# Autodesk Inventor assembly: Turntable-ArmConnection
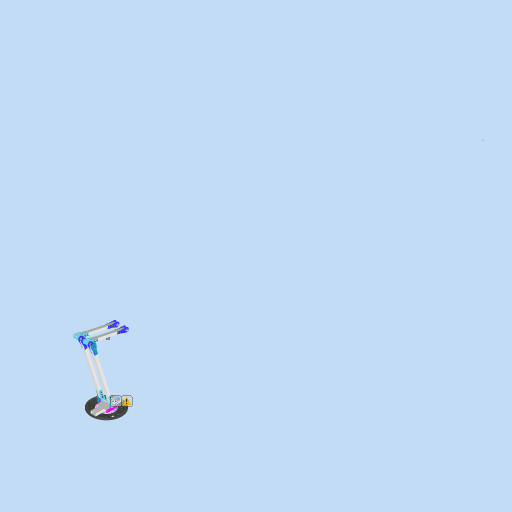
[picture p0: Inventor's stored thumbnail of the model, 512x512]
Saved by Autodesk Inventor 2024 (Build 280153000, 153)
## iProperties
Created: 2024-01-10
Part Number: Turntable-ArmConnection
Document SubType Name: Assembly
Designer: megan
Author: megan
## Documents named in this file (18)
- C:\Users\megan\OneDrive\Documents\GitHub\BehrendURCMechanical\CAD\Apparatus\Arm Base\Turntable-ArmConnection.iam
- C:\Users\megan\OneDrive\Documents\GitHub\BehrendURCMechanical\CAD\Apparatus\Arm Base\1544T3_Lubricated Turntable.ipt
- C:\Users\megan\OneDrive\Documents\GitHub\BehrendURCMechanical\CAD\Apparatus\Arm Base\2inTubeBase.ipt
- C:\Users\megan\OneDrive\Documents\GitHub\BehrendURCMechanical\CAD\Apparatus\Arm Base\1inTubeBase.ipt
- C:\Users\megan\OneDrive\Documents\GitHub\BehrendURCMechanical\CAD\Apparatus\Arm Base\ArmPlateBase.ipt
- C:\Users\megan\OneDrive\Documents\GitHub\BehrendURCMechanical\CAD\Apparatus\Arm Base\JointShaft.ipt
- C:\Users\megan\OneDrive\Documents\GitHub\BehrendURCMechanical\CAD\Chassis V3\Arm Plate2.ipt
- C:\Users\megan\OneDrive\Documents\GitHub\BehrendURCMechanical\CAD\Chassis V3\24in long 1in square tube.ipt
- C:\Users\megan\OneDrive\Documents\GitHub\BehrendURCMechanical\CAD\Chassis V3\Arm Plate3.ipt
- C:\Users\megan\OneDrive\Documents\GitHub\BehrendURCMechanical\CAD\Apparatus\Arm Base\8mmBearing.ipt
- C:\Users\megan\OneDrive\Documents\GitHub\BehrendURCMechanical\CAD\Chassis V3\Arm Plate.ipt
- C:\Users\megan\OneDrive\Documents\GitHub\BehrendURCMechanical\CAD\Chassis V3\14in long 1in square tube.ipt
- C:\Users\megan\OneDrive\Documents\GitHub\BehrendURCMechanical\CAD\Chassis V3\Bolt Nut Washer assem.iam
- C:\Users\megan\OneDrive\Documents\GitHub\BehrendURCMechanical\CAD\Apparatus\Arm Base\AP-0-02-baseAllTry2.iam
- C:\Users\megan\OneDrive\Documents\GitHub\BehrendURCMechanical\CAD\Chassis V3\90107A011_316 Stainless Steel Washer.ipt
- C:\Users\megan\OneDrive\Documents\GitHub\BehrendURCMechanical\CAD\Chassis V3\Arm Plate4.ipt
- C:\Users\megan\OneDrive\Documents\GitHub\BehrendURCMechanical\CAD\Apparatus\91290A198_Alloy Steel Socket Head Screw.ipt
- C:\Users\megan\OneDrive\Documents\GitHub\BehrendURCMechanical\CAD\Chassis V3\91831A011_18-8 Stainless Steel Nylon-Insert Locknut.ipt
## Components (75 placed, 14 different names)
1. 1544T3_Lubricated Turntable:1 — Mate:3, Mate:197, Mate:198, Mate:199, Mate:201
2. 2inTubeBase:1 — Mate:3, Mate:4, Mate:43, Mate:54, Mate:55, Mate:56, Flush:3, Flush:4, Flush:5, Mate:197, Mate:198
3. 1inTubeBase:1 — Mate:54, Mate:55, Mate:61, Mate:62, Flush:4
4. 1inTubeBase:2 — Mate:4, Mate:56, Flush:3, Mate:57, Mate:58, Mate:59, Mate:60
5. ArmPlateBase:2 — Mate:61, Mate:62, Flush:5, Mate:66
6. JointShaft:1 — Mate:22, Mate:33, Mate:36, Mate:37, Mate:63, Mate:83, Mate:84
7. arm plate:1 — Mate:22, Mate:34, Mate:73, Mate:74, Mate:142, Mate:143, Mate:150, Mate:151, Mate:152, Mate:153
8. ArmPlateBase:1 — Mate:57, Mate:58, Mate:59, Mate:60, Mate:63, Mate:65
9. 24in long 1in square tube:1 — Mate:44, Mate:45, Mate:46, Flush:2, Mate:67, Mate:68, Mate:69, Mate:70, Mate:71, Mate:72, Mate:86, Mate:200
10. 24in long 1in square tube:2 — Flush:2, Mate:49, Mate:50, Mate:51, Mate:73, Mate:74, Mate:85, Mate:204, Mate:207
11. arm plate:2 — Mate:33, Mate:34, Mate:43, Mate:44, Mate:45, Mate:46, Mate:144, Mate:145, Mate:146, Mate:147, Mate:148, Mate:149
12. 8mmBearing:1 — Mate:36, Mate:66
13. 8mmBearing:2 — Mate:37, Mate:65
14. arm plate:3 — Mate:80, Mate:81, Mate:204, Mate:207, Mate:236, Mate:237
15. arm plate:4 — Mate:49, Mate:50, Mate:51, Mate:213, Mate:262, Mate:264, Mate:266
16. arm plate:5 — Mate:67, Mate:68, Mate:69, Mate:77, Mate:78, Mate:154, Mate:155, Mate:156, Mate:157, Mate:158, Mate:168, Mate:169
17. arm plate:6 — Mate:70, Mate:71, Mate:72, Mate:79, Mate:82, Mate:161
18. 8mmBearing:4 — Mate:77, Mate:78, Mate:87
19. 8mmBearing:5 — Mate:79, Mate:82
20. 8mmBearing:6 — Mate:80, Mate:81, Mate:203, Mate:235
21. arm plate:7 — Mate:84, Mate:86
22. arm plate:8 — Mate:83, Mate:85
23. JointShaft:2 — Mate:87, Mate:93, Mate:95, Mate:97, Flush:10, Mate:203, Mate:212, Mate:226
24. 14in long 1in square tube:1 — Mate:101, Flush:7, Flush:8, Mate:106, Mate:107, Mate:110, Mate:115, Mate:116, Mate:159, Mate:227, Mate:228
25. 14in long 1in square tube:2 — Flush:8, Mate:103, Mate:104, Mate:105, Mate:108, Mate:109, Mate:112, Mate:113, Flush:9, Mate:114, Mate:160
26. arm plate:10 — Mate:93, Mate:104, Mate:105, Mate:161, Mate:170, Mate:171, Mate:172, Mate:173, Mate:174, Mate:175
27. arm plate:11 — Mate:95, Mate:101, Flush:7, Mate:158, Mate:159
28. arm plate:12 — Mate:97, Mate:103, Mate:160
29. arm plate:13 — Mate:106, Mate:107, Mate:111, Mate:115, Mate:117, Mate:124, Mate:188, Mate:189, Mate:190, Mate:191, Mate:192, Mate:193
30. arm plate:14 — Mate:108, Mate:109, Mate:114, Mate:122
31. arm plate:15 — Mate:110, Mate:111, Mate:116, Mate:120
32. arm plate:16 — Mate:112, Mate:113, Flush:9, Mate:118, Mate:182, Mate:183, Mate:184, Mate:185, Mate:186, Mate:187
33. JointShaft:3 — Mate:117, Flush:10, Mate:119, Mate:121, Mate:123, Mate:125, Flush:12
34. 8mmBearing:7 — Mate:124, Mate:125
35. 8mmBearing:8 — Mate:120, Mate:121
36. 8mmBearing:9 — Mate:118, Mate:119, Flush:12
37. 8mmBearing:10 — Mate:122, Mate:123
38. Bolt Nut Washer assem:1 [sub-assembly] — Mate:142, Mate:143
39. Bolt Nut Washer assem:2 [sub-assembly] — Mate:146, Mate:147
40. Bolt Nut Washer assem:3 [sub-assembly] — Mate:144, Mate:145
41. Bolt Nut Washer assem:4 [sub-assembly] — Mate:148, Mate:149
42. Bolt Nut Washer assem:5 [sub-assembly] — Mate:150, Mate:151
43. Bolt Nut Washer assem:6 [sub-assembly] — Mate:152, Mate:153
44. Bolt Nut Washer assem:7 [sub-assembly] — Mate:154, Mate:157
45. Bolt Nut Washer assem:8 [sub-assembly] — Mate:155, Mate:156
46. Bolt Nut Washer assem:9 [sub-assembly] — Mate:232, Mate:233
47. Bolt Nut Washer assem:10 [sub-assembly] — Mate:168, Mate:169
48. Bolt Nut Washer assem:11 [sub-assembly] — Mate:174, Mate:175
49. Bolt Nut Washer assem:13 [sub-assembly] — Mate:172, Mate:173
50. Bolt Nut Washer assem:14 [sub-assembly] — Mate:170, Mate:171
51. Bolt Nut Washer assem:15 [sub-assembly] — Mate:229, Mate:230
52. Bolt Nut Washer assem:16 [sub-assembly] — Mate:231, Mate:234
53. Bolt Nut Washer assem:17 [sub-assembly] — Mate:186, Mate:187
54. Bolt Nut Washer assem:18 [sub-assembly] — Mate:190, Mate:191
55. Bolt Nut Washer assem:19 [sub-assembly] — Mate:182, Mate:183
56. Bolt Nut Washer assem:20 [sub-assembly] — Mate:188, Mate:189
57. Bolt Nut Washer assem:21 [sub-assembly] — Mate:184, Mate:185
58. Bolt Nut Washer assem:24 [sub-assembly] — Mate:192, Mate:193
59. AP-0-02-baseAllTry2:1 [sub-assembly] — Mate:199
60. 8mmBearing:11 — Mate:212, Mate:213
61. 90107A011_316 Stainless Steel Washer:1 — Mate:240
62. 90107A011_316 Stainless Steel Washer:2 — Mate:246, Mate:247, Mate:250
63. 90107A011_316 Stainless Steel Washer:3 — Mate:243, Mate:244, Mate:245, Mate:246, Mate:249
64. arm plate:18 — Mate:226, Mate:227, Mate:228, Mate:229, Mate:230, Mate:231, Mate:232, Mate:233, Mate:234
65. arm plate:19 — Mate:235, Mate:236, Mate:237, Mate:240, Mate:243, Mate:244, Mate:245, Mate:247, Mate:248, Mate:251, Mate:252, Mate:253, Mate:255, Mate:256, Mate:258, Mate:260
66. 91290A198_Alloy Steel Socket Head Screw:1 — Mate:248, Mate:249, Mate:257, Mate:263
67. 91290A198_Alloy Steel Socket Head Screw:2 — Mate:254, Mate:255, Mate:261, Mate:267
68. 91290A198_Alloy Steel Socket Head Screw:3 — Mate:250, Mate:251, Mate:259, Mate:265
69. 90107A011_316 Stainless Steel Washer:4 — Mate:252, Mate:253, Mate:254
70. 91831A011_18-8 Stainless Steel Nylon-Insert Locknut:4 — Mate:256, Mate:257
71. 91831A011_18-8 Stainless Steel Nylon-Insert Locknut:5 — Mate:262, Mate:263
72. 91831A011_18-8 Stainless Steel Nylon-Insert Locknut:6 — Mate:260, Mate:261
73. 91831A011_18-8 Stainless Steel Nylon-Insert Locknut:7 — Mate:258, Mate:259
74. 91831A011_18-8 Stainless Steel Nylon-Insert Locknut:8 — Mate:266, Mate:267
75. 91831A011_18-8 Stainless Steel Nylon-Insert Locknut:9 — Mate:264, Mate:265
## Relationships (169: Mate 160, Flush 9)
- Mate:3: 1544T3_Lubricated Turntable:1 ↔ 2inTubeBase:1
- Mate:4: 2inTubeBase:1 ↔ 1inTubeBase:2
- Mate:22: JointShaft:1 ↔ arm plate:1
- Mate:33: JointShaft:1 ↔ arm plate:2
- Mate:34 (120.65 mm): arm plate:1 ↔ arm plate:2
- Mate:36: JointShaft:1 ↔ 8mmBearing:1
- Mate:37: JointShaft:1 ↔ 8mmBearing:2
- Mate:43 (60.325 mm): 2inTubeBase:1 ↔ arm plate:2
- Mate:44: 24in long 1in square tube:1 ↔ arm plate:2
- Mate:45: 24in long 1in square tube:1 ↔ arm plate:2
- Mate:46: 24in long 1in square tube:1 ↔ arm plate:2
- Flush:2: 24in long 1in square tube:1 ↔ 24in long 1in square tube:2
- Mate:49: 24in long 1in square tube:2 ↔ arm plate:4
- Mate:50: 24in long 1in square tube:2 ↔ arm plate:4
- Mate:51: 24in long 1in square tube:2 ↔ arm plate:4
- Mate:54: 2inTubeBase:1 ↔ 1inTubeBase:1
- Mate:55: 2inTubeBase:1 ↔ 1inTubeBase:1
- Mate:56: 2inTubeBase:1 ↔ 1inTubeBase:2
- Flush:3: 2inTubeBase:1 ↔ 1inTubeBase:2
- Mate:57: 1inTubeBase:2 ↔ ArmPlateBase:1
- Mate:58: 1inTubeBase:2 ↔ ArmPlateBase:1
- Mate:59: 1inTubeBase:2 ↔ ArmPlateBase:1
- Mate:60: 1inTubeBase:2 ↔ ArmPlateBase:1
- Mate:61: 1inTubeBase:1 ↔ ArmPlateBase:2
- Mate:62: 1inTubeBase:1 ↔ ArmPlateBase:2
- Flush:4: 2inTubeBase:1 ↔ 1inTubeBase:1
- Flush:5: 2inTubeBase:1 ↔ ArmPlateBase:2
- Mate:63: JointShaft:1 ↔ ArmPlateBase:1
- Mate:65: ArmPlateBase:1 ↔ 8mmBearing:2
- Mate:66: ArmPlateBase:2 ↔ 8mmBearing:1
- Mate:67: 24in long 1in square tube:1 ↔ arm plate:5
- Mate:68: 24in long 1in square tube:1 ↔ arm plate:5
- Mate:69: 24in long 1in square tube:1 ↔ arm plate:5
- Mate:70: 24in long 1in square tube:1 ↔ arm plate:6
- Mate:71: 24in long 1in square tube:1 ↔ arm plate:6
- Mate:72: 24in long 1in square tube:1 ↔ arm plate:6
- Mate:73: arm plate:1 ↔ 24in long 1in square tube:2
- Mate:74: arm plate:1 ↔ 24in long 1in square tube:2
- Mate:77: arm plate:5 ↔ 8mmBearing:4
- Mate:78: arm plate:5 ↔ 8mmBearing:4
- Mate:79: arm plate:6 ↔ 8mmBearing:5
- Mate:80: arm plate:3 ↔ 8mmBearing:6
- Mate:81: arm plate:3 ↔ 8mmBearing:6
- Mate:82: arm plate:6 ↔ 8mmBearing:5
- Mate:83: JointShaft:1 ↔ arm plate:8
- Mate:84: JointShaft:1 ↔ arm plate:7
- Mate:85: 24in long 1in square tube:2 ↔ arm plate:8
- Mate:86: 24in long 1in square tube:1 ↔ arm plate:7
- Mate:87: 8mmBearing:4 ↔ JointShaft:2
- Mate:93: JointShaft:2 ↔ arm plate:10
- Mate:95: JointShaft:2 ↔ arm plate:11
- Mate:97: JointShaft:2 ↔ arm plate:12
- Mate:101: 14in long 1in square tube:1 ↔ arm plate:11
- Flush:7: 14in long 1in square tube:1 ↔ arm plate:11
- Flush:8: 14in long 1in square tube:1 ↔ 14in long 1in square tube:2
- Mate:103: 14in long 1in square tube:2 ↔ arm plate:12
- Mate:104: 14in long 1in square tube:2 ↔ arm plate:10
- Mate:105: 14in long 1in square tube:2 ↔ arm plate:10
- Mate:106: 14in long 1in square tube:1 ↔ arm plate:13
- Mate:107: 14in long 1in square tube:1 ↔ arm plate:13
- Mate:108: 14in long 1in square tube:2 ↔ arm plate:14
- Mate:109: 14in long 1in square tube:2 ↔ arm plate:14
- Mate:110: 14in long 1in square tube:1 ↔ arm plate:15
- Mate:111: arm plate:13 ↔ arm plate:15
- Mate:112: 14in long 1in square tube:2 ↔ arm plate:16
- Mate:113: 14in long 1in square tube:2 ↔ arm plate:16
- Flush:9 (-2 mm): 14in long 1in square tube:2 ↔ arm plate:16
- Mate:114: 14in long 1in square tube:2 ↔ arm plate:14
- Mate:115: 14in long 1in square tube:1 ↔ arm plate:13
- Mate:116: 14in long 1in square tube:1 ↔ arm plate:15
- Mate:117: arm plate:13 ↔ JointShaft:3
- Flush:10: JointShaft:2 ↔ JointShaft:3
- Mate:118: arm plate:16 ↔ 8mmBearing:9
- Mate:119: JointShaft:3 ↔ 8mmBearing:9
- Mate:120: arm plate:15 ↔ 8mmBearing:8
- Mate:121: JointShaft:3 ↔ 8mmBearing:8
- Mate:122: arm plate:14 ↔ 8mmBearing:10
- Mate:123: JointShaft:3 ↔ 8mmBearing:10
- Mate:124: arm plate:13 ↔ 8mmBearing:7
- Mate:125: JointShaft:3 ↔ 8mmBearing:7
- Mate:142: arm plate:1 ↔ Bolt Nut Washer assem:1
- Mate:143: arm plate:1 ↔ Bolt Nut Washer assem:1
- Mate:144: arm plate:2 ↔ Bolt Nut Washer assem:3
- Mate:145: arm plate:2 ↔ Bolt Nut Washer assem:3
- Mate:146: arm plate:2 ↔ Bolt Nut Washer assem:2
- Mate:147: arm plate:2 ↔ Bolt Nut Washer assem:2
- Mate:148: arm plate:2 ↔ Bolt Nut Washer assem:4
- Mate:149: arm plate:2 ↔ Bolt Nut Washer assem:4
- Mate:150: arm plate:1 ↔ Bolt Nut Washer assem:5
- Mate:151: arm plate:1 ↔ Bolt Nut Washer assem:5
- Mate:152: arm plate:1 ↔ Bolt Nut Washer assem:6
- Mate:153: arm plate:1 ↔ Bolt Nut Washer assem:6
- Mate:154: arm plate:5 ↔ Bolt Nut Washer assem:7
- Mate:155: arm plate:5 ↔ Bolt Nut Washer assem:8
- Mate:156: arm plate:5 ↔ Bolt Nut Washer assem:8
- Mate:157: arm plate:5 ↔ Bolt Nut Washer assem:7
- Mate:158 (15.621 mm): arm plate:5 ↔ arm plate:11
- Mate:159: 14in long 1in square tube:1 ↔ arm plate:11
- Mate:160: 14in long 1in square tube:2 ↔ arm plate:12
- Mate:161 (15.621 mm): arm plate:6 ↔ arm plate:10
- Mate:168: arm plate:5 ↔ Bolt Nut Washer assem:10
- Mate:169: arm plate:5 ↔ Bolt Nut Washer assem:10
- Mate:170: arm plate:10 ↔ Bolt Nut Washer assem:14
- Mate:171: arm plate:10 ↔ Bolt Nut Washer assem:14
- Mate:172: arm plate:10 ↔ Bolt Nut Washer assem:13
- Mate:173: arm plate:10 ↔ Bolt Nut Washer assem:13
- Mate:174: arm plate:10 ↔ Bolt Nut Washer assem:11
- Mate:175: arm plate:10 ↔ Bolt Nut Washer assem:11
- Mate:182: arm plate:16 ↔ Bolt Nut Washer assem:19
- Mate:183: arm plate:16 ↔ Bolt Nut Washer assem:19
- Mate:184: arm plate:16 ↔ Bolt Nut Washer assem:21
- Mate:185: arm plate:16 ↔ Bolt Nut Washer assem:21
- Mate:186: arm plate:16 ↔ Bolt Nut Washer assem:17
- Mate:187: arm plate:16 ↔ Bolt Nut Washer assem:17
- Mate:188: arm plate:13 ↔ Bolt Nut Washer assem:20
- Mate:189: arm plate:13 ↔ Bolt Nut Washer assem:20
- Mate:190: arm plate:13 ↔ Bolt Nut Washer assem:18
- Mate:191: arm plate:13 ↔ Bolt Nut Washer assem:18
- Mate:192: arm plate:13 ↔ Bolt Nut Washer assem:24
- Mate:193: arm plate:13 ↔ Bolt Nut Washer assem:24
- Mate:197: 1544T3_Lubricated Turntable:1 ↔ 2inTubeBase:1
- Mate:198: 1544T3_Lubricated Turntable:1 ↔ 2inTubeBase:1
- Mate:199: 1544T3_Lubricated Turntable:1 ↔ AP-0-02-baseAllTry2:1
- Mate:200: 24in long 1in square tube:1
- Mate:201: 1544T3_Lubricated Turntable:1
- Mate:203: 8mmBearing:6 ↔ JointShaft:2
- Mate:204: 24in long 1in square tube:2 ↔ arm plate:3
- Mate:207: 24in long 1in square tube:2 ↔ arm plate:3
- Mate:212: JointShaft:2 ↔ 8mmBearing:11
- Mate:213: arm plate:4 ↔ 8mmBearing:11
- Flush:12 (-12.7 mm): JointShaft:3 ↔ 8mmBearing:9
- Mate:226: JointShaft:2 ↔ arm plate:18
- Mate:227: 14in long 1in square tube:1 ↔ arm plate:18
- Mate:228: 14in long 1in square tube:1 ↔ arm plate:18
- Mate:229: Bolt Nut Washer assem:15 ↔ arm plate:18
- Mate:230: Bolt Nut Washer assem:15 ↔ arm plate:18
- Mate:231: Bolt Nut Washer assem:16 ↔ arm plate:18
- Mate:232: Bolt Nut Washer assem:9 ↔ arm plate:18
- Mate:233: Bolt Nut Washer assem:9 ↔ arm plate:18
- Mate:234: Bolt Nut Washer assem:16 ↔ arm plate:18
- Mate:235: 8mmBearing:6 ↔ arm plate:19
- Mate:236 (6.35 mm): arm plate:3 ↔ arm plate:19
- Mate:237: arm plate:3 ↔ arm plate:19
- Mate:240: 90107A011_316 Stainless Steel Washer:1 ↔ arm plate:19
- Mate:243: 90107A011_316 Stainless Steel Washer:3 ↔ arm plate:19
- Mate:244: 90107A011_316 Stainless Steel Washer:3 ↔ arm plate:19
- Mate:245: 90107A011_316 Stainless Steel Washer:3 ↔ arm plate:19
- Mate:246: 90107A011_316 Stainless Steel Washer:2 ↔ 90107A011_316 Stainless Steel Washer:3
- Mate:247: 90107A011_316 Stainless Steel Washer:2 ↔ arm plate:19
- Mate:248: arm plate:19 ↔ 91290A198_Alloy Steel Socket Head Screw:1
- Mate:249: 90107A011_316 Stainless Steel Washer:3 ↔ 91290A198_Alloy Steel Socket Head Screw:1
- Mate:250: 90107A011_316 Stainless Steel Washer:2 ↔ 91290A198_Alloy Steel Socket Head Screw:3
- Mate:251: arm plate:19 ↔ 91290A198_Alloy Steel Socket Head Screw:3
- Mate:252: arm plate:19 ↔ 90107A011_316 Stainless Steel Washer:4
- Mate:253: arm plate:19 ↔ 90107A011_316 Stainless Steel Washer:4
- Mate:254: 91290A198_Alloy Steel Socket Head Screw:2 ↔ 90107A011_316 Stainless Steel Washer:4
- Mate:255: arm plate:19 ↔ 91290A198_Alloy Steel Socket Head Screw:2
- Mate:256: arm plate:19 ↔ 91831A011_18-8 Stainless Steel Nylon-Insert Locknut:4
- Mate:257: 91290A198_Alloy Steel Socket Head Screw:1 ↔ 91831A011_18-8 Stainless Steel Nylon-Insert Locknut:4
- Mate:258: arm plate:19 ↔ 91831A011_18-8 Stainless Steel Nylon-Insert Locknut:7
- Mate:259: 91290A198_Alloy Steel Socket Head Screw:3 ↔ 91831A011_18-8 Stainless Steel Nylon-Insert Locknut:7
- Mate:260: arm plate:19 ↔ 91831A011_18-8 Stainless Steel Nylon-Insert Locknut:6
- Mate:261: 91290A198_Alloy Steel Socket Head Screw:2 ↔ 91831A011_18-8 Stainless Steel Nylon-Insert Locknut:6
- Mate:262: arm plate:4 ↔ 91831A011_18-8 Stainless Steel Nylon-Insert Locknut:5
- Mate:263: 91290A198_Alloy Steel Socket Head Screw:1 ↔ 91831A011_18-8 Stainless Steel Nylon-Insert Locknut:5
- Mate:264: arm plate:4 ↔ 91831A011_18-8 Stainless Steel Nylon-Insert Locknut:9
- Mate:265: 91290A198_Alloy Steel Socket Head Screw:3 ↔ 91831A011_18-8 Stainless Steel Nylon-Insert Locknut:9
- Mate:266: arm plate:4 ↔ 91831A011_18-8 Stainless Steel Nylon-Insert Locknut:8
- Mate:267: 91290A198_Alloy Steel Socket Head Screw:2 ↔ 91831A011_18-8 Stainless Steel Nylon-Insert Locknut:8
